# Autodesk Inventor assembly: coverslip_holder_body_only_assembly
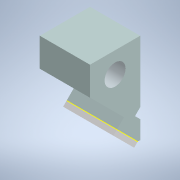
[picture p0: Inventor's stored thumbnail of the model, 180x180]
Saved by Autodesk Inventor 2022 (Build 260153000, 153)
## iProperties
Created: 2021-10-05
Part Number: coverslip_holder_body_only_assembly
Document SubType Name: Assembly
Designer: Spectral
Author: Spectral
## Documents named in this file (3)
- C:\Users\Spectral\Documents\GitHub\manuscripts\2021-dean-protocol\cad\coverslip_holder_body_only_assembly.iam
- C:\Users\Spectral\Documents\GitHub\manuscripts\2021-dean-protocol\cad\coverslip_holder_body_only.ipt
- C:\Users\Spectral\Documents\GitHub\manuscripts\2021-dean-protocol\cad\coverslip_holder_bracket.ipt
## Components (2 placed, 2 different names)
1. coverslip_holder_body_only:1 — Mate:1, Flush:1, Flush:2
2. coverslip_holder_bracket:1 — Mate:1, Flush:1, Flush:2
## Relationships (3: Flush 2, Mate 1)
- Mate:1: coverslip_holder_body_only:1 ↔ coverslip_holder_bracket:1
- Flush:1: coverslip_holder_body_only:1 ↔ coverslip_holder_bracket:1
- Flush:2: coverslip_holder_body_only:1 ↔ coverslip_holder_bracket:1
